# Autodesk Inventor assembly: Stepper with wheel
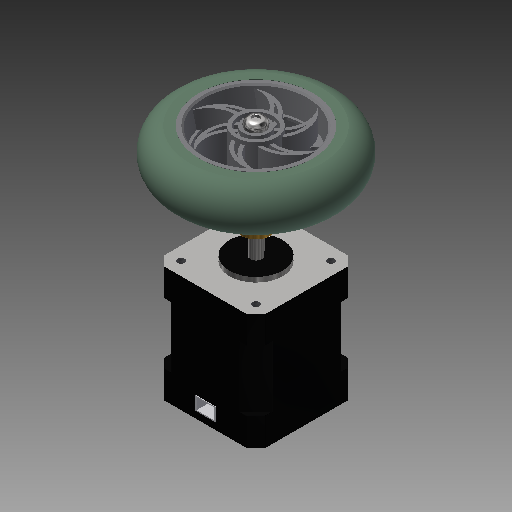
[picture p0: Inventor's stored thumbnail of the model, 512x512]
Saved by Autodesk Inventor 2018 (Build 220112000, 112)
## iProperties
Created: 2018-05-02
Part Number: Stepper with wheel
Document SubType Name: Assembly
Designer: Ajith Thomas
Author: Ajith Thomas
## Documents named in this file (5)
- C:\Users\Ajith Thomas\Dropbox\Gas_Sensing_Robot\FumeBot-Design\Stepper with wheel.iam
- C:\Users\Ajith Thomas\Dropbox\Gas_Sensing_Robot\FumeBot-Design\Stepper Motor\Stepper.iam
- C:\Users\Ajith Thomas\Dropbox\Gas_Sensing_Robot\FumeBot-Design\Wheel Coupler.ipt
- C:\Users\Ajith Thomas\Dropbox\Gas_Sensing_Robot\FumeBot-Design\Wheel.ipt
- C:\Users\Ajith Thomas\Dropbox\Gas_Sensing_Robot\FumeBot-Design\Wheel coupler screw.ipt
## Components (4 placed, 4 different names)
1. Stepper:1 [sub-assembly] — Mate:4, Mate:5, Angle:1
2. Wheel Coupler:1 — Mate:2, Mate:3, Mate:4, Mate:5, Angle:1, Angle:2
3. Wheel:1 — Mate:2, Mate:3, Angle:2, Mate:6, Mate:7
4. Wheel coupler screw:1 — Mate:6, Mate:7
## Relationships (8: Mate 6, Angle 2)
- Mate:2: Wheel Coupler:1 ↔ Wheel:1
- Mate:3: Wheel Coupler:1 ↔ Wheel:1
- Mate:4: Stepper:1 ↔ Wheel Coupler:1
- Mate:5: Stepper:1 ↔ Wheel Coupler:1
- Angle:1 (0 deg): Stepper:1 ↔ Wheel Coupler:1
- Angle:2 (0 deg): Wheel Coupler:1 ↔ Wheel:1
- Mate:6: Wheel:1 ↔ Wheel coupler screw:1
- Mate:7: Wheel:1 ↔ Wheel coupler screw:1
